# Autodesk Inventor assembly: 45 deg with session mount for boolian
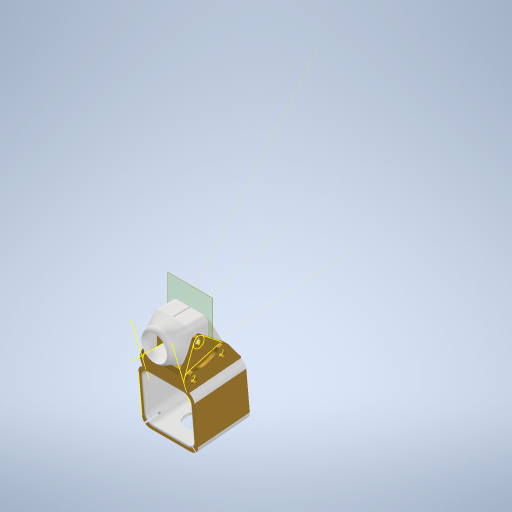
[picture p0: Inventor's stored thumbnail of the model, 512x512]
Saved by Autodesk Inventor 2023 (Build 270158000, 158)
## iProperties
Created: 2023-02-19
Part Number: 45 deg with session mount for boolian
Document SubType Name: Assembly
Designer: Steven
Author: Steven
## Documents named in this file (3)
- Y:\FPV drone stuff\0 Street League\Frames\PB-Kauri-X\3D prints\35 mm canopy\work in progress prints\Camera mounts\predator mini\45 deg with session mount for boolian.iam
- Y:\FPV drone stuff\0 Street League\Frames\PB-Kauri-X\3D prints\35 mm canopy\work in progress prints\Camera mounts\predator mini\45 deg mini predator fixed mount.ipt
- Y:\FPV drone stuff\0 Street League\Frames\PB-Kauri-X\3D prints\35 mm canopy\work in progress prints\session mounts\V2 session mount 45deg block.ipt
## Components (2 placed, 2 different names)
1. 45 deg mini predator fixed mount:1 — Mate:1, Mate:2, Mate:3
2. V2 session mount 45deg block:1 — Mate:1, Mate:2, Mate:3
## Relationships (3: Mate 3)
- Mate:1: 45 deg mini predator fixed mount:1 ↔ V2 session mount 45deg block:1
- Mate:2: 45 deg mini predator fixed mount:1 ↔ V2 session mount 45deg block:1
- Mate:3 (2.2 mm): 45 deg mini predator fixed mount:1 ↔ V2 session mount 45deg block:1
